# Autodesk Inventor assembly: VertWeaponMount
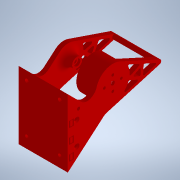
[picture p0: Inventor's stored thumbnail of the model, 180x180]
Saved by Autodesk Inventor 2020 (Build 240168000, 168)
## iProperties
Created: 2024-02-06
Part Number: VertWeaponMount
Document SubType Name: Assembly
Designer: smz3rm
Mass: 55.0409 g
Surface Area: 321.616 cm^2
Volume: 55.0409 cm^3
Density: 1 g/cm^3
Author: smz3rm
## Documents named in this file (5)
- C:\Users\smz3rm\OneDrive - BP\Documents\Battlebots\VerticalSpinner\VertWeaponMount.iam
- C:\Users\smz3rm\OneDrive - BP\Documents\Battlebots\VerticalSpinner\WeaponMountBaseV1.ipt
- C:\Users\smz3rm\OneDrive - BP\Documents\Battlebots\VerticalSpinner\WeaponMountLeftPlateV1.ipt
- C:\Users\smz3rm\OneDrive - BP\Documents\Battlebots\VerticalSpinner\WeaponMountRightPlateV1.ipt
- C:\Users\smz3rm\OneDrive - BP\Documents\Battlebots\VerticalSpinner\WeaponMountBasePlateV1.ipt
## Components (3 placed, 3 different names)
1. WeaponMountBaseV1:1 — Mate:1, Mate:2, Mate:3, Mate:4, Mate:5, Mate:6, Flush:1, Flush:2, Mate:9, Mate:10, Mate:11, Mate:12
2. WeaponMountLeftPlateV1:1 — Mate:1, Mate:3, Mate:4, Flush:2, Mate:11, Mate:12
3. WeaponMountRightPlateV1:1 — Mate:2, Mate:5, Mate:6, Flush:1, Mate:9, Mate:10
## Relationships (12: Mate 10, Flush 2)
- Mate:1: WeaponMountBaseV1:1 ↔ WeaponMountLeftPlateV1:1
- Mate:2: WeaponMountBaseV1:1 ↔ WeaponMountRightPlateV1:1
- Mate:3 (0.4 mm): WeaponMountBaseV1:1 ↔ WeaponMountLeftPlateV1:1
- Mate:4 (0.4 mm): WeaponMountBaseV1:1 ↔ WeaponMountLeftPlateV1:1
- Mate:5 (0.4 mm): WeaponMountBaseV1:1 ↔ WeaponMountRightPlateV1:1
- Mate:6 (0.4 mm): WeaponMountBaseV1:1 ↔ WeaponMountRightPlateV1:1
- Flush:1: WeaponMountBaseV1:1 ↔ WeaponMountRightPlateV1:1
- Flush:2: WeaponMountBaseV1:1 ↔ WeaponMountLeftPlateV1:1
- Mate:9 (0.4 mm): WeaponMountBaseV1:1 ↔ WeaponMountRightPlateV1:1
- Mate:10 (0.4 mm): WeaponMountBaseV1:1 ↔ WeaponMountRightPlateV1:1
- Mate:11: WeaponMountBaseV1:1 ↔ WeaponMountLeftPlateV1:1
- Mate:12: WeaponMountBaseV1:1 ↔ WeaponMountLeftPlateV1:1
## Named parameters: SlotTolerance = 0.8 mm
